# Autodesk Inventor assembly: airhockeybot_mechanical
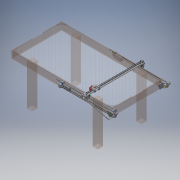
[picture p0: Inventor's stored thumbnail of the model, 180x180]
Saved by Autodesk Inventor 2019.3 (Build 233278000, 278)
## iProperties
Created: 2020-08-23
Part Number: airhockeybot_mechanical
Material: Generisch
Document SubType Name: Assembly
Designer: Nicolas Frick
Author: Nicolas Frick
## Documents named in this file (46)
- C:\Users\Nicolas Frick\Sync\OneDrive\airhockeybot\mechanical_design\inventor\airhockeybot_mechanical.iam
- C:\Users\Nicolas Frick\Sync\OneDrive\airhockeybot\mechanical_design\inventor\Table\Table.iam
- C:\Users\Nicolas Frick\Sync\OneDrive\airhockeybot\mechanical_design\inventor\Pulley.iam
- C:\Users\Nicolas Frick\Sync\OneDrive\airhockeybot\mechanical_design\inventor\Fixture_mid.ipt
- C:\Users\Nicolas Frick\Sync\OneDrive\airhockeybot\mechanical_design\inventor\Fixture_linear_mid.ipt
- C:\Users\Nicolas Frick\Sync\OneDrive\airhockeybot\mechanical_design\inventor\Bearing_support_outside.ipt
- C:\Users\Nicolas Frick\Sync\OneDrive\airhockeybot\mechanical_design\inventor\Bearing_support_inside.ipt
- C:\Users\Nicolas Frick\Sync\OneDrive\airhockeybot\mechanical_design\inventor\igus\EEWM_12_200_2.ipt
- C:\Users\Nicolas Frick\Sync\OneDrive\airhockeybot\mechanical_design\inventor\igus\RJUM_01_12_3.ipt
- C:\Users\Nicolas Frick\Sync\OneDrive\airhockeybot\mechanical_design\inventor\Switch CMV101D\CNDT_CMV101D.ipt
- C:\Users\Nicolas Frick\Sync\OneDrive\airhockeybot\mechanical_design\inventor\PowerS.ipt
- C:\Users\Nicolas Frick\Sync\OneDrive\airhockeybot\mechanical_design\inventor\PowerS_case.ipt
- C:\Users\Nicolas Frick\Sync\OneDrive\airhockeybot\mechanical_design\inventor\Cable_clamp.ipt
- C:\Users\Nicolas Frick\Sync\OneDrive\airhockeybot\mechanical_design\inventor\PowerS_cap.ipt
- C:\Users\Nicolas Frick\Sync\OneDrive\airhockeybot\mechanical_design\inventor\Nema 17HS5425\Assembly1.iam
- C:\Users\Nicolas Frick\Sync\OneDrive\airhockeybot\mechanical_design\inventor\GT2 40T 5mm Bore 6mm wide pulley\GT2 40T 5 Bore v2.iam
- C:\Users\Nicolas Frick\Sync\OneDrive\airhockeybot\mechanical_design\inventor\Fixture_linear_end.ipt
- C:\Users\Nicolas Frick\Sync\OneDrive\airhockeybot\mechanical_design\inventor\Fixture_motor.ipt
- C:\Users\Nicolas Frick\Sync\OneDrive\airhockeybot\mechanical_design\inventor\bat.ipt
- C:\Users\Nicolas Frick\Sync\OneDrive\airhockeybot\mechanical_design\inventor\igus\WS_10_40_200_2_modify.ipt
- C:\Users\Nicolas Frick\Sync\OneDrive\airhockeybot\mechanical_design\inventor\igus\Schlitten_WW_10_40_10_1.ipt
- C:\Users\Nicolas Frick\Sync\OneDrive\airhockeybot\mechanical_design\inventor\GT2 Belt 6mm\GT2 Belt 6mm x 40mm.ipt
- C:\Users\Nicolas Frick\Sync\OneDrive\airhockeybot\mechanical_design\inventor\Fixture_mid_right.ipt
- C:\Users\Nicolas Frick\Sync\OneDrive\airhockeybot\mechanical_design\inventor\Fixture_linear_mid_right.ipt
- C:\Users\Nicolas Frick\Sync\OneDrive\airhockeybot\mechanical_design\inventor\Fixture_motor_right.ipt
- C:\Users\Nicolas Frick\Sync\OneDrive\airhockeybot\mechanical_design\inventor\Fixture_linear_end_right.ipt
- C:\Users\Nicolas Frick\Sync\OneDrive\airhockeybot\mechanical_design\inventor\bat_handle.ipt
- C:\Users\Nicolas Frick\Sync\OneDrive\airhockeybot\mechanical_design\inventor\Upper_left_fixture.ipt
- C:\Users\Nicolas Frick\Sync\OneDrive\airhockeybot\mechanical_design\inventor\Belt_clamp.ipt
- C:\Users\Nicolas Frick\Sync\OneDrive\airhockeybot\mechanical_design\inventor\Belt_clamp_mirrored.ipt
- C:\Users\Nicolas Frick\Sync\OneDrive\airhockeybot\mechanical_design\inventor\Distance_lin.ipt
- C:\Users\Nicolas Frick\Sync\OneDrive\airhockeybot\mechanical_design\inventor\Upper_right_fixture.ipt
- C:\Users\Nicolas Frick\Sync\OneDrive\airhockeybot\mechanical_design\inventor\Upper_bearing_support_inside.ipt
- C:\Users\Nicolas Frick\Sync\OneDrive\airhockeybot\mechanical_design\inventor\Upper_bearing_support_outside.ipt
- C:\Users\Nicolas Frick\Sync\OneDrive\airhockeybot\mechanical_design\inventor\Chain\chain.iam
- C:\Users\Nicolas Frick\Sync\OneDrive\airhockeybot\mechanical_design\inventor\Chain\chain_end_elmt.ipt
- C:\Users\Nicolas Frick\Sync\OneDrive\airhockeybot\mechanical_design\inventor\Chain_fixture.ipt
- C:\Users\Nicolas Frick\Sync\OneDrive\airhockeybot\mechanical_design\inventor\Bat_fixture.ipt
- C:\Users\Nicolas Frick\Sync\OneDrive\airhockeybot\mechanical_design\inventor\MaedlerKlemmplatte_T2_5_6mm\16069900.ipt
- C:\Users\Nicolas Frick\Sync\OneDrive\airhockeybot\mechanical_design\inventor\Bat_claw.ipt
- C:\Users\Nicolas Frick\Sync\OneDrive\airhockeybot\mechanical_design\inventor\Pusher.ipt
- C:\Users\Nicolas Frick\Sync\OneDrive\airhockeybot\mechanical_design\inventor\Stiff_motor.ipt
- C:\Users\Nicolas Frick\Sync\OneDrive\airhockeybot\mechanical_design\inventor\beam.ipt
- C:\Users\Nicolas Frick\Sync\OneDrive\airhockeybot\mechanical_design\inventor\Chain_support.ipt
- C:\Users\Nicolas Frick\Sync\OneDrive\airhockeybot\mechanical_design\inventor\Stiff.ipt
- C:\Users\Nicolas Frick\Sync\OneDrive\airhockeybot\mechanical_design\inventor\Table\Plate.ipt
## Components (244 placed, 45 different names)
1. Table:1 [sub-assembly] — Fluchtend:1, Passend:1, Passend:2, Passend:5, Fluchtend:2, Fluchtend:3, Fluchtend:4, Passend:36, Passend:37, Passend:42, Passend:43, Fluchtend:26, Passend:69, Passend:70, Passend:86, Passend:87, Passend:203, Passend:204, Passend:209, Passend:210, Passend:211
2. Fixture_mid:1 — Fluchtend:1, Passend:1, Passend:2, Passend:3, Passend:4, Passend:6, Passend:7, Fluchtend:27, Fluchtend:28
3. Fixture_linear_mid:1 — Passend:3, Passend:4, Passend:5, Passend:23, Fluchtend:6
4. Bearing_support_outside:1 — Passend:10, Passend:11, Passend:12, Fluchtend:15, Passend:62, Passend:65, Fluchtend:25, Passend:66
5. Bearing_support_inside:1 — Passend:6, Passend:7, Passend:10, Passend:11, Passend:12, Fluchtend:24, Passend:63, Passend:67
6. EEWM_12_200_2:1 — Passend:17, Passend:18, Passend:41, Passend:114, Fluchtend:72
7. RJUM_01_12_3:1 — Passend:17, Passend:108, Fluchtend:37, Passend:115
8. RJUM_01_12_3:2 — Passend:18, Passend:107, Fluchtend:36
9. CNDT_CMV101D:1 — Passend:23, Fluchtend:6
10. PowerS:1 — Fluchtend:8, Fluchtend:11, Fluchtend:12, Passend:36, Passend:37
11. PowerS_case:1 — Fluchtend:8, Passend:31, Fluchtend:9, Fluchtend:10, Passend:32, Passend:33, Passend:34, Fluchtend:11, Fluchtend:12, Passend:212
12. Cable_clamp:1 — Passend:31, Fluchtend:9, Fluchtend:10
13. PowerS_cap:1 — Passend:32, Passend:33, Passend:34
14. Assembly1:1 [sub-assembly] — Passend:38, Fluchtend:15, Passend:44, Passend:58, Passend:68
15. GT2 40T 5 Bore v2:1 [sub-assembly] — Passend:38, Passend:68
16. Fixture_linear_end:1 — Passend:39, Fluchtend:17, Passend:41, Passend:46, Fluchtend:19, Fluchtend:22, Passend:59, Fluchtend:72
17. Fixture_motor:1 — Passend:39, Fluchtend:17, Passend:42, Passend:43, Passend:44, Passend:58, Passend:59, Fluchtend:29, Passend:176, Fluchtend:62, Fluchtend:82
18. CNDT_CMV101D:2 — Passend:46, Fluchtend:19, Fluchtend:22
19. bat:1 — Passend:98, Passend:99, Passend:213
20. WS_10_40_200_2_modify:1 — Passend:52, Passend:53, Passend:54, Passend:187, Passend:188, Passend:189
21. Schlitten_WW_10_40_10_1:1 — Passend:52, Passend:53, Passend:54, Fluchtend:64, Passend:179, Passend:180, Passend:181, Passend:182
22. Pulley:1 [sub-assembly] — Passend:66, Passend:67
23. Fixture_mid_right:1 — Passend:69, Fluchtend:27, Fluchtend:28, Passend:71, Passend:72, Passend:73, Passend:75
24. Fixture_linear_mid_right:1 — Passend:70, Passend:71, Passend:72, Passend:186
25. Bearing_support_inside:2 — Passend:73, Passend:75, Passend:77, Passend:78, Passend:79, Passend:81, Passend:101, Passend:103, Fluchtend:34
26. Bearing_support_outside:2 — Passend:78, Passend:80, Passend:81, Passend:100, Fluchtend:33, Passend:102
27. Pulley:2 [sub-assembly] — Passend:77, Passend:79, Passend:80
28. EEWM_12_200_2:2 — Passend:82, Passend:83, Passend:88, Passend:120, Passend:186, Fluchtend:71
29. RJUM_01_12_3:3 — Passend:82, Passend:118, Passend:121, Fluchtend:45
30. RJUM_01_12_3:4 — Passend:83, Passend:119, Passend:122
31. Fixture_motor_right:1 — Passend:86, Fluchtend:29, Passend:87, Passend:89, Passend:90, Passend:95, Passend:96, Passend:104
32. Fixture_linear_end_right:1 — Passend:88, Passend:89, Passend:90, Fluchtend:71
33. Assembly1:2 [sub-assembly] — Passend:95, Passend:96, Passend:97, Fluchtend:32, Passend:104
34. GT2 40T 5 Bore v2:2 [sub-assembly] — Passend:97, Fluchtend:32
35. bat_handle:1 — Passend:98, Passend:99, Passend:184
36. Upper_left_fixture:1 — Passend:107, Passend:108, Fluchtend:36, Fluchtend:37, Fluchtend:38, Fluchtend:39, Fluchtend:40, Fluchtend:44, Passend:146, Passend:147, Passend:187, Passend:189, Passend:191, Fluchtend:75, Fluchtend:76, Passend:199, Passend:200, Fluchtend:80
37. Assembly1:3 [sub-assembly] — Passend:105, Passend:106, Fluchtend:38, Fluchtend:39, Fluchtend:40
38. GT2 40T 5 Bore v2:3 [sub-assembly] — Passend:105, Passend:106
39. Belt_clamp:1 — Passend:110, Passend:111, Fluchtend:41, Fluchtend:42, Passend:147, Passend:195, Passend:197, Passend:198
40. Belt_clamp_mirrored:1 — Fluchtend:41, Fluchtend:42, Passend:146
41. Distance_lin:1 — Passend:114, Passend:115
42. Upper_right_fixture:1 — Fluchtend:44, Passend:118, Passend:119, Fluchtend:45, Passend:131, Passend:132, Passend:144, Passend:145, Passend:188, Passend:192, Passend:193
43. Distance_lin:2 — Passend:120, Passend:121, Passend:122
44. Upper_bearing_support_inside:1 — Passend:127, Passend:128, Fluchtend:48, Fluchtend:49, Passend:130, Passend:131, Passend:132
45. Pulley:3 [sub-assembly] — Passend:127, Passend:128, Passend:129
46. Upper_bearing_support_outside:1 — Fluchtend:48, Fluchtend:49, Passend:129, Passend:130, Passend:140, Passend:141, Fluchtend:52, Passend:142, Passend:143, Fluchtend:53
47. Belt_clamp:2 — Fluchtend:50, Fluchtend:51, Passend:144, Passend:206, Passend:208
48. Belt_clamp_mirrored:2 — Passend:134, Passend:135, Fluchtend:50, Fluchtend:51, Passend:145, Passend:207
49. chain_end_elmt:1 — Passend:170, Fluchtend:56, Passend:199, Passend:200, Fluchtend:80
50. chain_end_elmt:2 — Passend:201, Fluchtend:81, Passend:202, Fluchtend:82
51. chain:27 [sub-assembly] — Passend:162, Passend:163, Passend:164, Passend:167
52. chain:28 [sub-assembly] — Passend:165, Passend:166, Passend:168, Passend:169
53. chain:29 [sub-assembly] — Passend:164, Passend:165, Passend:166, Passend:167
54. chain:30 [sub-assembly] — Passend:158, Passend:159, Passend:160, Passend:161
55. chain:31 [sub-assembly] — Passend:160, Passend:161, Passend:162, Passend:163
56. chain:32 [sub-assembly] — Passend:156, Passend:157, Passend:158, Passend:159
57. chain:33 [sub-assembly] — Passend:156, Passend:157, Passend:170, Fluchtend:56
58. Chain_fixture:1 — Passend:176, Fluchtend:62, Passend:202
59. Bat_fixture:1 — Fluchtend:64, Fluchtend:65, Fluchtend:67, Fluchtend:68, Passend:178, Passend:181, Passend:182, Fluchtend:69, Fluchtend:70, Passend:185, Fluchtend:77, Fluchtend:85, Fluchtend:86
60. 16069900:1 — Fluchtend:65, Fluchtend:67, Passend:180
61. 16069900:2 — Fluchtend:68, Passend:178, Passend:179
62. Bat_claw:1 — Fluchtend:69, Fluchtend:70, Passend:184, Passend:185
63. CNDT_CMV101D:6 — Passend:191, Fluchtend:75, Fluchtend:76
64. Pusher:1 — Fluchtend:77, Fluchtend:85, Fluchtend:86
65. CNDT_CMV101D:7 — Passend:192, Passend:193
66. Stiff_motor:1 — Passend:195, Passend:197, Passend:198
67. beam:1 — Passend:203, Fluchtend:83, Passend:204, Fluchtend:84
68. Chain_support:1 — Fluchtend:84
69. Stiff:1 — Passend:206, Passend:207, Passend:208
70. Plate:1 — Passend:209, Passend:210, Passend:211, Passend:212, Passend:213
71. GT2 Belt 6mm x 40mm:1 — Fluchtend:24, Passend:63
72. GT2 Belt 6mm x 40mm:2 — Passend:62
73. GT2 Belt 6mm x 40mm:3
74. GT2 Belt 6mm x 40mm:4
75. GT2 Belt 6mm x 40mm:5
76. GT2 Belt 6mm x 40mm:6
77. GT2 Belt 6mm x 40mm:7
78. GT2 Belt 6mm x 40mm:8
79. GT2 Belt 6mm x 40mm:9
80. GT2 Belt 6mm x 40mm:10
81. GT2 Belt 6mm x 40mm:11
82. GT2 Belt 6mm x 40mm:12
83. GT2 Belt 6mm x 40mm:13
84. GT2 Belt 6mm x 40mm:14
85. GT2 Belt 6mm x 40mm:15
86. GT2 Belt 6mm x 40mm:16
87. GT2 Belt 6mm x 40mm:17
88. GT2 Belt 6mm x 40mm:18
89. GT2 Belt 6mm x 40mm:19
90. GT2 Belt 6mm x 40mm:20
91. GT2 Belt 6mm x 40mm:21
92. GT2 Belt 6mm x 40mm:22 — Passend:110, Passend:111
93. GT2 Belt 6mm x 40mm:23
94. GT2 Belt 6mm x 40mm:24
95. GT2 Belt 6mm x 40mm:25 — Passend:65, Fluchtend:25
96. GT2 Belt 6mm x 40mm:26
97. GT2 Belt 6mm x 40mm:27
98. GT2 Belt 6mm x 40mm:28
99. GT2 Belt 6mm x 40mm:29
100. GT2 Belt 6mm x 40mm:30
101. GT2 Belt 6mm x 40mm:31
102. GT2 Belt 6mm x 40mm:32 — Fluchtend:26
103. GT2 Belt 6mm x 40mm:33
104. GT2 Belt 6mm x 40mm:34
105. GT2 Belt 6mm x 40mm:35
106. GT2 Belt 6mm x 40mm:36
107. GT2 Belt 6mm x 40mm:37
108. GT2 Belt 6mm x 40mm:38
109. GT2 Belt 6mm x 40mm:39
110. GT2 Belt 6mm x 40mm:40
111. GT2 Belt 6mm x 40mm:41
112. GT2 Belt 6mm x 40mm:42
113. GT2 Belt 6mm x 40mm:43
114. GT2 Belt 6mm x 40mm:44
115. GT2 Belt 6mm x 40mm:45
116. GT2 Belt 6mm x 40mm:46
117. GT2 Belt 6mm x 40mm:47
118. GT2 Belt 6mm x 40mm:48
119. GT2 Belt 6mm x 40mm:49 — Passend:100, Passend:101, Fluchtend:33
120. GT2 Belt 6mm x 40mm:51
121. GT2 Belt 6mm x 40mm:52
122. GT2 Belt 6mm x 40mm:53
123. GT2 Belt 6mm x 40mm:54
124. GT2 Belt 6mm x 40mm:55
125. GT2 Belt 6mm x 40mm:56
126. GT2 Belt 6mm x 40mm:57
127. GT2 Belt 6mm x 40mm:58
128. GT2 Belt 6mm x 40mm:59
129. GT2 Belt 6mm x 40mm:60
130. GT2 Belt 6mm x 40mm:61
131. GT2 Belt 6mm x 40mm:62
132. GT2 Belt 6mm x 40mm:63
133. GT2 Belt 6mm x 40mm:64
134. GT2 Belt 6mm x 40mm:65
135. GT2 Belt 6mm x 40mm:66
136. GT2 Belt 6mm x 40mm:67
137. GT2 Belt 6mm x 40mm:68
138. GT2 Belt 6mm x 40mm:69
139. GT2 Belt 6mm x 40mm:70
140. GT2 Belt 6mm x 40mm:71 — Passend:134, Passend:135
141. GT2 Belt 6mm x 40mm:72
142. GT2 Belt 6mm x 40mm:73
143. GT2 Belt 6mm x 40mm:50 — Passend:102, Passend:103, Fluchtend:34
144. GT2 Belt 6mm x 40mm:74
145. GT2 Belt 6mm x 40mm:75
146. GT2 Belt 6mm x 40mm:76
147. GT2 Belt 6mm x 40mm:77
148. GT2 Belt 6mm x 40mm:78
149. GT2 Belt 6mm x 40mm:79
150. GT2 Belt 6mm x 40mm:80
151. GT2 Belt 6mm x 40mm:81
152. GT2 Belt 6mm x 40mm:82
153. GT2 Belt 6mm x 40mm:83
154. GT2 Belt 6mm x 40mm:84
155. GT2 Belt 6mm x 40mm:85
156. GT2 Belt 6mm x 40mm:86
157. GT2 Belt 6mm x 40mm:87
158. GT2 Belt 6mm x 40mm:88
159. GT2 Belt 6mm x 40mm:89
160. GT2 Belt 6mm x 40mm:90
161. GT2 Belt 6mm x 40mm:91
162. GT2 Belt 6mm x 40mm:92
163. GT2 Belt 6mm x 40mm:93
164. GT2 Belt 6mm x 40mm:94
165. GT2 Belt 6mm x 40mm:95
166. GT2 Belt 6mm x 40mm:96
167. GT2 Belt 6mm x 40mm:98 — Passend:140, Passend:141, Fluchtend:52
168. GT2 Belt 6mm x 40mm:99
169. GT2 Belt 6mm x 40mm:100
170. GT2 Belt 6mm x 40mm:101
171. GT2 Belt 6mm x 40mm:102
172. GT2 Belt 6mm x 40mm:103
173. GT2 Belt 6mm x 40mm:104
174. GT2 Belt 6mm x 40mm:105
175. GT2 Belt 6mm x 40mm:106
176. GT2 Belt 6mm x 40mm:107
177. GT2 Belt 6mm x 40mm:108
178. GT2 Belt 6mm x 40mm:109
179. GT2 Belt 6mm x 40mm:110
180. GT2 Belt 6mm x 40mm:111
181. GT2 Belt 6mm x 40mm:112
182. GT2 Belt 6mm x 40mm:113
183. GT2 Belt 6mm x 40mm:114
184. GT2 Belt 6mm x 40mm:115
185. GT2 Belt 6mm x 40mm:116
186. GT2 Belt 6mm x 40mm:117
187. GT2 Belt 6mm x 40mm:118
188. GT2 Belt 6mm x 40mm:119
189. GT2 Belt 6mm x 40mm:120
190. GT2 Belt 6mm x 40mm:121
191. GT2 Belt 6mm x 40mm:122
192. GT2 Belt 6mm x 40mm:123
193. GT2 Belt 6mm x 40mm:97 — Passend:142, Passend:143, Fluchtend:53
194. GT2 Belt 6mm x 40mm:124
195. GT2 Belt 6mm x 40mm:125
196. GT2 Belt 6mm x 40mm:126
197. GT2 Belt 6mm x 40mm:127
198. GT2 Belt 6mm x 40mm:128
199. GT2 Belt 6mm x 40mm:129
200. GT2 Belt 6mm x 40mm:130
201. GT2 Belt 6mm x 40mm:131
202. GT2 Belt 6mm x 40mm:132
203. GT2 Belt 6mm x 40mm:133
204. GT2 Belt 6mm x 40mm:134
205. GT2 Belt 6mm x 40mm:135
206. GT2 Belt 6mm x 40mm:136
207. GT2 Belt 6mm x 40mm:137
208. GT2 Belt 6mm x 40mm:138
209. GT2 Belt 6mm x 40mm:139
210. GT2 Belt 6mm x 40mm:140
211. GT2 Belt 6mm x 40mm:141
212. GT2 Belt 6mm x 40mm:142
213. GT2 Belt 6mm x 40mm:143
214. GT2 Belt 6mm x 40mm:144
215. GT2 Belt 6mm x 40mm:145
216. GT2 Belt 6mm x 40mm:146
217. GT2 Belt 6mm x 40mm:147
218. GT2 Belt 6mm x 40mm:148
219. chain:1 [sub-assembly] — Passend:201, Fluchtend:81
220. chain:2 [sub-assembly]
221. chain:3 [sub-assembly]
222. chain:4 [sub-assembly]
223. chain:5 [sub-assembly]
224. chain:6 [sub-assembly]
225. chain:7 [sub-assembly]
226. chain:8 [sub-assembly] — Fluchtend:83
227. chain:9 [sub-assembly]
228. chain:10 [sub-assembly]
229. chain:11 [sub-assembly]
230. chain:12 [sub-assembly]
231. chain:13 [sub-assembly]
232. chain:14 [sub-assembly]
233. chain:15 [sub-assembly]
234. chain:16 [sub-assembly]
235. chain:17 [sub-assembly]
236. chain:18 [sub-assembly]
237. chain:19 [sub-assembly]
238. chain:20 [sub-assembly]
239. chain:21 [sub-assembly]
240. chain:22 [sub-assembly]
241. chain:23 [sub-assembly]
242. chain:24 [sub-assembly]
243. chain:25 [sub-assembly]
244. chain:26 [sub-assembly] — Passend:168, Passend:169
## Component patterns: (24 elements, first: GT2 Belt 6mm x 40mm:1), (24 elements, first: GT2 Belt 6mm x 40mm:25), (24 elements, first: GT2 Belt 6mm x 40mm:49), (24 elements, first: GT2 Belt 6mm x 40mm:50), (26 elements, first: GT2 Belt 6mm x 40mm:98), (26 elements, first: GT2 Belt 6mm x 40mm:97), (26 elements, first: chain:1)
## Relationships (199: Mate 141, Flush 58)
- Fluchtend:1 [Flush] (747.832 mm): Table:1 ↔ Fixture_mid:1
- Passend:1 [Mate]: Table:1 ↔ Fixture_mid:1
- Passend:2 [Mate] (74 mm): Table:1 ↔ Fixture_mid:1
- Passend:3 [Mate]: Fixture_mid:1 ↔ Fixture_linear_mid:1
- Passend:4 [Mate]: Fixture_mid:1 ↔ Fixture_linear_mid:1
- Passend:5 [Mate]: Table:1 ↔ Fixture_linear_mid:1
- Fluchtend:2 [Flush]: Table:1
- Fluchtend:3 [Flush]: Table:1
- Fluchtend:4 [Flush]: Table:1
- Passend:6 [Mate] (0.05 mm): Fixture_mid:1 ↔ Bearing_support_inside:1
- Passend:7 [Mate] (0.05 mm): Fixture_mid:1 ↔ Bearing_support_inside:1
- Passend:10 [Mate]: Bearing_support_outside:1 ↔ Bearing_support_inside:1
- Passend:11 [Mate]: Bearing_support_outside:1 ↔ Bearing_support_inside:1
- Passend:12 [Mate]: Bearing_support_outside:1 ↔ Bearing_support_inside:1
- Passend:17 [Mate]: EEWM_12_200_2:1 ↔ RJUM_01_12_3:1
- Passend:18 [Mate]: EEWM_12_200_2:1 ↔ RJUM_01_12_3:2
- Passend:23 [Mate]: Fixture_linear_mid:1 ↔ CNDT_CMV101D:1
- Fluchtend:6 [Flush]: Fixture_linear_mid:1 ↔ CNDT_CMV101D:1
- Fluchtend:8 [Flush]: PowerS:1 ↔ PowerS_case:1
- Passend:31 [Mate]: PowerS_case:1 ↔ Cable_clamp:1
- Fluchtend:9 [Flush]: PowerS_case:1 ↔ Cable_clamp:1
- Fluchtend:10 [Flush]: PowerS_case:1 ↔ Cable_clamp:1
- Passend:32 [Mate]: PowerS_case:1 ↔ PowerS_cap:1
- Passend:33 [Mate]: PowerS_case:1 ↔ PowerS_cap:1
- Passend:34 [Mate]: PowerS_case:1 ↔ PowerS_cap:1
- Fluchtend:11 [Flush]: PowerS:1 ↔ PowerS_case:1
- Fluchtend:12 [Flush]: PowerS:1 ↔ PowerS_case:1
- Passend:36 [Mate] (50 mm): Table:1 ↔ PowerS:1
- Passend:37 [Mate] (250 mm): Table:1 ↔ PowerS:1
- Passend:38 [Mate]: Assembly1:1 ↔ GT2 40T 5 Bore v2:1
- Fluchtend:15 [Flush] (3.85 mm): Bearing_support_outside:1 ↔ Assembly1:1
- Passend:39 [Mate]: Fixture_linear_end:1 ↔ Fixture_motor:1
- Fluchtend:17 [Flush]: Fixture_linear_end:1 ↔ Fixture_motor:1
- Passend:41 [Mate]: EEWM_12_200_2:1 ↔ Fixture_linear_end:1
- Passend:42 [Mate]: Table:1 ↔ Fixture_motor:1
- Passend:43 [Mate]: Table:1 ↔ Fixture_motor:1
- Passend:44 [Mate]: Assembly1:1 ↔ Fixture_motor:1
- Passend:46 [Mate]: Fixture_linear_end:1 ↔ CNDT_CMV101D:2
- Fluchtend:19 [Flush] (12 mm): Fixture_linear_end:1 ↔ CNDT_CMV101D:2
- Passend:52 [Mate]: WS_10_40_200_2_modify:1 ↔ Schlitten_WW_10_40_10_1:1
- Passend:53 [Mate]: WS_10_40_200_2_modify:1 ↔ Schlitten_WW_10_40_10_1:1
- Passend:54 [Mate]: WS_10_40_200_2_modify:1 ↔ Schlitten_WW_10_40_10_1:1
- Passend:58 [Mate] (0.15 mm): Assembly1:1 ↔ Fixture_motor:1
- Fluchtend:22 [Flush] (4 mm): Fixture_linear_end:1 ↔ CNDT_CMV101D:2
- Passend:59 [Mate]: Fixture_linear_end:1 ↔ Fixture_motor:1
- Passend:62 [Mate] (2.7 mm): Bearing_support_outside:1 ↔ GT2 Belt 6mm x 40mm:2
- Fluchtend:24 [Flush] (16.1 mm): Bearing_support_inside:1 ↔ GT2 Belt 6mm x 40mm:1
- Passend:63 [Mate] (12.7 mm): Bearing_support_inside:1 ↔ GT2 Belt 6mm x 40mm:1
- Passend:65 [Mate] (5.5 mm): Bearing_support_outside:1 ↔ GT2 Belt 6mm x 40mm:25
- Fluchtend:25 [Flush] (15 mm): Bearing_support_outside:1 ↔ GT2 Belt 6mm x 40mm:25
- Fluchtend:26 [Flush] (52 mm): Table:1 ↔ GT2 Belt 6mm x 40mm:32
- Passend:66 [Mate]: Bearing_support_outside:1 ↔ Pulley:1
- Passend:67 [Mate]: Bearing_support_inside:1 ↔ Pulley:1
- Passend:68 [Mate] (2.5 mm): Assembly1:1 ↔ GT2 40T 5 Bore v2:1
- Passend:69 [Mate]: Table:1 ↔ Fixture_mid_right:1
- Fluchtend:27 [Flush]: Fixture_mid:1 ↔ Fixture_mid_right:1
- Fluchtend:28 [Flush]: Fixture_mid:1 ↔ Fixture_mid_right:1
- Passend:70 [Mate]: Table:1 ↔ Fixture_linear_mid_right:1
- Passend:71 [Mate]: Fixture_mid_right:1 ↔ Fixture_linear_mid_right:1
- Passend:72 [Mate]: Fixture_mid_right:1 ↔ Fixture_linear_mid_right:1
- Passend:73 [Mate]: Fixture_mid_right:1 ↔ Bearing_support_inside:2
- Passend:75 [Mate] (0.1 mm): Fixture_mid_right:1 ↔ Bearing_support_inside:2
- Passend:77 [Mate]: Bearing_support_inside:2 ↔ Pulley:2
- Passend:78 [Mate]: Bearing_support_inside:2 ↔ Bearing_support_outside:2
- Passend:79 [Mate]: Bearing_support_inside:2 ↔ Pulley:2
- Passend:80 [Mate]: Bearing_support_outside:2 ↔ Pulley:2
- Passend:81 [Mate]: Bearing_support_inside:2 ↔ Bearing_support_outside:2
- Passend:82 [Mate]: EEWM_12_200_2:2 ↔ RJUM_01_12_3:3
- Passend:83 [Mate]: EEWM_12_200_2:2 ↔ RJUM_01_12_3:4
- Passend:86 [Mate]: Table:1 ↔ Fixture_motor_right:1
- Fluchtend:29 [Flush]: Fixture_motor:1 ↔ Fixture_motor_right:1
- Passend:87 [Mate]: Table:1 ↔ Fixture_motor_right:1
- Passend:88 [Mate]: EEWM_12_200_2:2 ↔ Fixture_linear_end_right:1
- Passend:89 [Mate]: Fixture_motor_right:1 ↔ Fixture_linear_end_right:1
- Passend:90 [Mate]: Fixture_motor_right:1 ↔ Fixture_linear_end_right:1
- Passend:95 [Mate]: Fixture_motor_right:1 ↔ Assembly1:2
- Passend:96 [Mate]: Fixture_motor_right:1 ↔ Assembly1:2
- Passend:97 [Mate]: Assembly1:2 ↔ GT2 40T 5 Bore v2:2
- Fluchtend:32 [Flush] (-3 mm): Assembly1:2 ↔ GT2 40T 5 Bore v2:2
- Passend:98 [Mate]: bat:1 ↔ bat_handle:1
- Passend:99 [Mate]: bat:1 ↔ bat_handle:1
- Passend:100 [Mate] (2.5 mm): Bearing_support_outside:2 ↔ GT2 Belt 6mm x 40mm:49
- Passend:101 [Mate] (12.8 mm): Bearing_support_inside:2 ↔ GT2 Belt 6mm x 40mm:49
- Fluchtend:33 [Flush] (20 mm): Bearing_support_outside:2 ↔ GT2 Belt 6mm x 40mm:49
- Passend:102 [Mate] (2.5 mm): Bearing_support_outside:2 ↔ GT2 Belt 6mm x 40mm:50
- Passend:103 [Mate] (12.8 mm): Bearing_support_inside:2 ↔ GT2 Belt 6mm x 40mm:50
- Fluchtend:34 [Flush] (20 mm): Bearing_support_inside:2 ↔ GT2 Belt 6mm x 40mm:50
- Passend:104 [Mate] (3.984 mm): Fixture_motor_right:1 ↔ Assembly1:2
- Passend:105 [Mate]: Assembly1:3 ↔ GT2 40T 5 Bore v2:3
- Passend:106 [Mate] (1.3 mm): Assembly1:3 ↔ GT2 40T 5 Bore v2:3
- Passend:107 [Mate]: RJUM_01_12_3:2 ↔ Upper_left_fixture:1
- Passend:108 [Mate]: RJUM_01_12_3:1 ↔ Upper_left_fixture:1
- Fluchtend:36 [Flush]: RJUM_01_12_3:2 ↔ Upper_left_fixture:1
- Fluchtend:37 [Flush]: RJUM_01_12_3:1 ↔ Upper_left_fixture:1
- Fluchtend:38 [Flush] (13 mm): Upper_left_fixture:1 ↔ Assembly1:3
- Fluchtend:39 [Flush] (5 mm): Upper_left_fixture:1 ↔ Assembly1:3
- Fluchtend:40 [Flush] (10 mm): Upper_left_fixture:1 ↔ Assembly1:3
- Passend:110 [Mate] (0.5 mm): Belt_clamp:1 ↔ GT2 Belt 6mm x 40mm:22
- Passend:111 [Mate] (1 mm): Belt_clamp:1 ↔ GT2 Belt 6mm x 40mm:22
- Fluchtend:41 [Flush]: Belt_clamp:1 ↔ Belt_clamp_mirrored:1
- Fluchtend:42 [Flush]: Belt_clamp:1 ↔ Belt_clamp_mirrored:1
- Passend:114 [Mate]: EEWM_12_200_2:1 ↔ Distance_lin:1
- Passend:115 [Mate]: RJUM_01_12_3:1 ↔ Distance_lin:1
- Fluchtend:44 [Flush]: Upper_left_fixture:1 ↔ Upper_right_fixture:1
- Passend:118 [Mate]: RJUM_01_12_3:3 ↔ Upper_right_fixture:1
- Passend:119 [Mate]: RJUM_01_12_3:4 ↔ Upper_right_fixture:1
- Passend:120 [Mate]: EEWM_12_200_2:2 ↔ Distance_lin:2
- Passend:121 [Mate]: RJUM_01_12_3:3 ↔ Distance_lin:2
- Passend:122 [Mate]: RJUM_01_12_3:4 ↔ Distance_lin:2
- Fluchtend:45 [Flush]: RJUM_01_12_3:3 ↔ Upper_right_fixture:1
- Passend:127 [Mate]: Upper_bearing_support_inside:1 ↔ Pulley:3
- Passend:128 [Mate]: Upper_bearing_support_inside:1 ↔ Pulley:3
- Fluchtend:48 [Flush]: Upper_bearing_support_inside:1 ↔ Upper_bearing_support_outside:1
- Fluchtend:49 [Flush]: Upper_bearing_support_inside:1 ↔ Upper_bearing_support_outside:1
- Passend:129 [Mate]: Pulley:3 ↔ Upper_bearing_support_outside:1
- Passend:130 [Mate]: Upper_bearing_support_inside:1 ↔ Upper_bearing_support_outside:1
- Passend:131 [Mate] (0.1 mm): Upper_right_fixture:1 ↔ Upper_bearing_support_inside:1
- Passend:132 [Mate]: Upper_right_fixture:1 ↔ Upper_bearing_support_inside:1
- Passend:134 [Mate] (1 mm): Belt_clamp_mirrored:2 ↔ GT2 Belt 6mm x 40mm:71
- Passend:135 [Mate] (0.2 mm): Belt_clamp_mirrored:2 ↔ GT2 Belt 6mm x 40mm:71
- Fluchtend:50 [Flush]: Belt_clamp:2 ↔ Belt_clamp_mirrored:2
- Fluchtend:51 [Flush]: Belt_clamp:2 ↔ Belt_clamp_mirrored:2
- Passend:140 [Mate] (2.5 mm): Upper_bearing_support_outside:1 ↔ GT2 Belt 6mm x 40mm:98
- Passend:141 [Mate] (5.4 mm): Upper_bearing_support_outside:1 ↔ GT2 Belt 6mm x 40mm:98
- Fluchtend:52 [Flush] (20 mm): Upper_bearing_support_outside:1 ↔ GT2 Belt 6mm x 40mm:98
- Passend:142 [Mate] (2.5 mm): Upper_bearing_support_outside:1 ↔ GT2 Belt 6mm x 40mm:97
- Passend:143 [Mate] (5.5 mm): Upper_bearing_support_outside:1 ↔ GT2 Belt 6mm x 40mm:97
- Fluchtend:53 [Flush] (20 mm): Upper_bearing_support_outside:1 ↔ GT2 Belt 6mm x 40mm:97
- Passend:144 [Mate]: Upper_right_fixture:1 ↔ Belt_clamp:2
- Passend:145 [Mate]: Upper_right_fixture:1 ↔ Belt_clamp_mirrored:2
- Passend:146 [Mate]: Upper_left_fixture:1 ↔ Belt_clamp_mirrored:1
- Passend:147 [Mate]: Upper_left_fixture:1 ↔ Belt_clamp:1
- Passend:156 [Mate]: chain:32 ↔ chain:33
- Passend:157 [Mate]: chain:32 ↔ chain:33
- Passend:158 [Mate]: chain:30 ↔ chain:32
- Passend:159 [Mate]: chain:30 ↔ chain:32
- Passend:160 [Mate]: chain:30 ↔ chain:31
- Passend:161 [Mate]: chain:30 ↔ chain:31
- Passend:162 [Mate]: chain:27 ↔ chain:31
- Passend:163 [Mate]: chain:27 ↔ chain:31
- Passend:164 [Mate]: chain:27 ↔ chain:29
- Passend:165 [Mate]: chain:28 ↔ chain:29
- Passend:166 [Mate]: chain:28 ↔ chain:29
- Passend:167 [Mate]: chain:27 ↔ chain:29
- Passend:168 [Mate]: chain:28 ↔ chain:26
- Passend:169 [Mate]: chain:28 ↔ chain:26
- Passend:170 [Mate]: chain_end_elmt:1 ↔ chain:33
- Fluchtend:56 [Flush] (-1 mm): chain_end_elmt:1 ↔ chain:33
- Passend:176 [Mate]: Fixture_motor:1 ↔ Chain_fixture:1
- Fluchtend:62 [Flush]: Fixture_motor:1 ↔ Chain_fixture:1
- Fluchtend:64 [Flush]: Schlitten_WW_10_40_10_1:1 ↔ Bat_fixture:1
- Fluchtend:65 [Flush] (-5.5 mm): Bat_fixture:1 ↔ 16069900:1
- Fluchtend:67 [Flush] (20 mm): Bat_fixture:1 ↔ 16069900:1
- Fluchtend:68 [Flush] (-5.5 mm): Bat_fixture:1 ↔ 16069900:2
- Passend:178 [Mate]: Bat_fixture:1 ↔ 16069900:2
- Passend:179 [Mate]: Schlitten_WW_10_40_10_1:1 ↔ 16069900:2
- Passend:180 [Mate]: Schlitten_WW_10_40_10_1:1 ↔ 16069900:1
- Passend:181 [Mate]: Schlitten_WW_10_40_10_1:1 ↔ Bat_fixture:1
- Passend:182 [Mate]: Schlitten_WW_10_40_10_1:1 ↔ Bat_fixture:1
- Fluchtend:69 [Flush] (30 mm): Bat_fixture:1 ↔ Bat_claw:1
- Fluchtend:70 [Flush]: Bat_fixture:1 ↔ Bat_claw:1
- Passend:184 [Mate]: bat_handle:1 ↔ Bat_claw:1
- Passend:185 [Mate]: Bat_fixture:1 ↔ Bat_claw:1
- Passend:186 [Mate]: Fixture_linear_mid_right:1 ↔ EEWM_12_200_2:2
- Fluchtend:71 [Flush]: EEWM_12_200_2:2 ↔ Fixture_linear_end_right:1
- Fluchtend:72 [Flush]: EEWM_12_200_2:1 ↔ Fixture_linear_end:1
- Passend:187 [Mate]: WS_10_40_200_2_modify:1 ↔ Upper_left_fixture:1
- Passend:188 [Mate]: WS_10_40_200_2_modify:1 ↔ Upper_right_fixture:1
- Passend:189 [Mate]: WS_10_40_200_2_modify:1 ↔ Upper_left_fixture:1
- Passend:191 [Mate]: Upper_left_fixture:1 ↔ CNDT_CMV101D:6
- Fluchtend:75 [Flush] (1 mm): Upper_left_fixture:1 ↔ CNDT_CMV101D:6
- Fluchtend:76 [Flush] (4 mm): Upper_left_fixture:1 ↔ CNDT_CMV101D:6
- Fluchtend:77 [Flush]: Bat_fixture:1 ↔ Pusher:1
- Passend:192 [Mate]: Upper_right_fixture:1 ↔ CNDT_CMV101D:7
- Passend:193 [Mate]: Upper_right_fixture:1 ↔ CNDT_CMV101D:7
- Passend:195 [Mate]: Belt_clamp:1 ↔ Stiff_motor:1
- Passend:197 [Mate]: Belt_clamp:1 ↔ Stiff_motor:1
- Passend:198 [Mate]: Belt_clamp:1 ↔ Stiff_motor:1
- Passend:199 [Mate]: Upper_left_fixture:1 ↔ chain_end_elmt:1
- Passend:200 [Mate] (-17 mm): Upper_left_fixture:1 ↔ chain_end_elmt:1
- Fluchtend:80 [Flush]: Upper_left_fixture:1 ↔ chain_end_elmt:1
- Passend:201 [Mate]: chain_end_elmt:2 ↔ chain:1
- Fluchtend:81 [Flush] (-1 mm): chain_end_elmt:2 ↔ chain:1
- Passend:202 [Mate]: chain_end_elmt:2 ↔ Chain_fixture:1
- Fluchtend:82 [Flush]: Fixture_motor:1 ↔ chain_end_elmt:2
- Passend:203 [Mate]: Table:1 ↔ beam:1
- Fluchtend:83 [Flush]: beam:1 ↔ chain:8
- Passend:204 [Mate] (80 mm): Table:1 ↔ beam:1
- Fluchtend:84 [Flush]: beam:1 ↔ Chain_support:1
- Passend:206 [Mate]: Belt_clamp:2 ↔ Stiff:1
- Passend:207 [Mate]: Belt_clamp_mirrored:2 ↔ Stiff:1
- Passend:208 [Mate]: Belt_clamp:2 ↔ Stiff:1
- Passend:209 [Mate]: Table:1 ↔ Plate:1
- Passend:210 [Mate]: Table:1 ↔ Plate:1
- Passend:211 [Mate]: Table:1 ↔ Plate:1
- Passend:212 [Mate]: PowerS_case:1 ↔ Plate:1
- Passend:213 [Mate]: bat:1 ↔ Plate:1
- Fluchtend:85 [Flush] (-10 mm): Bat_fixture:1 ↔ Pusher:1
- Fluchtend:86 [Flush] (2 mm): Bat_fixture:1 ↔ Pusher:1
